# Autodesk Inventor assembly: mosaad pump
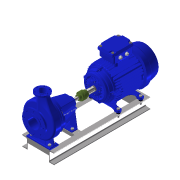
[picture p0: Inventor's stored thumbnail of the model, 180x180]
Saved by Autodesk Inventor 2016 (Build 200138000, 138)
## iProperties
Created: 2017-06-04
Part Number: mosaad pump
Document SubType Name: Assembly
Designer: Mohamed
Author: Mohamed
## Documents named in this file (12)
- C:\Users\Mohamed\Desktop\Mosaad pump\mosaad pump.iam
- C:\Users\Mohamed\Desktop\Mosaad pump\nnnnmmm.ipt
- C:\Users\Mohamed\Desktop\Mosaad pump\Assembly3.iam
- C:\Users\Mohamed\Desktop\Mosaad pump\DIN1026-1 - U 60 - 350.ipt
- C:\Users\Mohamed\Desktop\Mosaad pump\DIN1026-1 - U 80 - 350.ipt
- C:\Users\Mohamed\Desktop\Mosaad pump\rubber.ipt
- C:\Users\Mohamed\Documents\Inventor\Content Center Files\R2016\en-US\DIN 1026-1\DIN1026-1 - U 100 - 900.ipt
- C:\Users\Mohamed\Documents\Inventor\Content Center Files\R2016\en-US\DIN 933\DIN 933 - M14  x 65.ipt
- C:\Users\Mohamed\Documents\Inventor\Content Center Files\R2016\en-US\DIN 934\DIN 934 - M14 x 2.ipt
- C:\Users\Mohamed\Documents\Inventor\Content Center Files\R2016\en-US\DIN 1026-1\DIN1026-1 - U 100 - 200.ipt
- C:\Users\Mohamed\Desktop\Mosaad pump\coupling1.ipt
- C:\Users\Mohamed\Desktop\Mosaad pump\coupling2.ipt
## Components (27 placed, 11 different names)
1. nnnnmmm:1 — Mate:3, Angle:1, Mate:11, Mate:13, Mate:17, Mate:18, Mate:30, Mate:31, Mate:32, Mate:33, Mate:34, Mate:35, Mate:39, Mate:57, Mate:58
2. Assembly3:1 [sub-assembly] — Mate:3, Flush:6, Flush:8, Angle:1, Mate:24, Mate:25, Mate:41, Mate:42, Mate:43, Mate:44, Mate:45, Mate:46, Mate:47, Mate:48, Mate:49, Mate:50, Mate:51, Mate:52, Mate:59, Mate:60
3. DIN1026-1 - U 60 - 350:2 — Flush:7, Flush:8, Flush:12, Mate:27
4. DIN1026-1 - U 80 - 350:1 — Flush:6, Flush:7, Mate:22, Flush:13, Mate:24, Mate:26
5. rubber:1 — Mate:11, Mate:35
6. rubber:2 — Mate:17, Mate:33, Mate:54
7. rubber:3 — Mate:18, Mate:34, Mate:56
8. rubber:4 — Mate:13, Mate:32
9. DIN 1026-1 U 100 - 900:1 — Mate:26, Flush:14, Flush:15, Mate:40
10. DIN 1026-1 U 100 - 900:2 — Mate:22, Flush:12, Flush:13, Mate:23, Mate:25, Flush:14, Flush:15, Mate:27, Mate:36, Flush:18, Flush:19, Flush:24, Flush:25
11. DIN 933 - replaced by DIN EN 24017 M14  x 65:1 — Mate:30, Mate:31, Mate:37, Flush:16, Flush:20
12. DIN 934 - replaced by DIN EN 24032/28673/28674 M14:1 — Mate:36, Mate:37, Flush:17, Flush:21
13. DIN 933 - replaced by DIN EN 24017 M14  x 65:2 — Flush:16, Mate:39
14. DIN 934 - replaced by DIN EN 24032/28673/28674 M14:2 — Flush:17
15. DIN 1026-1 U 100 - 200:1 — Mate:40, Flush:18, Flush:19
16. DIN 933 - replaced by DIN EN 24017 M14  x 65:3 — Mate:41, Mate:42
17. DIN 933 - replaced by DIN EN 24017 M14  x 65:4 — Mate:43, Mate:44
18. DIN 933 - replaced by DIN EN 24017 M14  x 65:5 — Mate:45, Mate:46
19. DIN 933 - replaced by DIN EN 24017 M14  x 65:6 — Mate:47, Mate:48
20. DIN 933 - replaced by DIN EN 24017 M14  x 65:7 — Mate:49, Mate:50
21. DIN 933 - replaced by DIN EN 24017 M14  x 65:8 — Mate:51, Mate:52
22. DIN 933 - replaced by DIN EN 24017 M14  x 65:9 — Mate:54, Flush:20, Flush:23
23. DIN 934 - replaced by DIN EN 24032/28673/28674 M14:3 — Flush:21, Flush:22
24. DIN 933 - replaced by DIN EN 24017 M14  x 65:10 — Mate:56, Flush:23
25. DIN 934 - replaced by DIN EN 24032/28673/28674 M14:4 — Flush:22
26. coupling1:1 — Mate:57, Mate:58, Mate:61, Mate:62
27. coupling2:1 — Mate:59, Mate:60, Mate:61, Mate:62
## Relationships (62: Mate 44, Flush 17, Angle 1)
- Mate:3: nnnnmmm:1 ↔ Assembly3:1
- Flush:6: Assembly3:1 ↔ DIN1026-1 - U 80 - 350:1
- Flush:7: DIN1026-1 - U 60 - 350:2 ↔ DIN1026-1 - U 80 - 350:1
- Flush:8 (-3 mm): Assembly3:1 ↔ DIN1026-1 - U 60 - 350:2
- Angle:1 (0 deg): nnnnmmm:1 ↔ Assembly3:1
- Mate:11: nnnnmmm:1 ↔ rubber:1
- Mate:13: nnnnmmm:1 ↔ rubber:4
- Mate:17: nnnnmmm:1 ↔ rubber:2
- Mate:18: nnnnmmm:1 ↔ rubber:3
- Mate:22: DIN1026-1 - U 80 - 350:1 ↔ DIN 1026-1 U 100 - 900:2
- Flush:12: DIN1026-1 - U 60 - 350:2 ↔ DIN 1026-1 U 100 - 900:2
- Flush:13: DIN1026-1 - U 80 - 350:1 ↔ DIN 1026-1 U 100 - 900:2
- Mate:23: DIN 1026-1 U 100 - 900:2
- Mate:24: Assembly3:1 ↔ DIN1026-1 - U 80 - 350:1
- Mate:25 (-10 mm): Assembly3:1 ↔ DIN 1026-1 U 100 - 900:2
- Mate:26: DIN1026-1 - U 80 - 350:1 ↔ DIN 1026-1 U 100 - 900:1
- Flush:14: DIN 1026-1 U 100 - 900:1 ↔ DIN 1026-1 U 100 - 900:2
- Flush:15: DIN 1026-1 U 100 - 900:1 ↔ DIN 1026-1 U 100 - 900:2
- Mate:27: DIN1026-1 - U 60 - 350:2 ↔ DIN 1026-1 U 100 - 900:2
- Mate:30: nnnnmmm:1 ↔ DIN 933 - replaced by DIN EN 24017 M14  x 65:1
- Mate:31: nnnnmmm:1 ↔ DIN 933 - replaced by DIN EN 24017 M14  x 65:1
- Mate:32: nnnnmmm:1 ↔ rubber:4
- Mate:33: nnnnmmm:1 ↔ rubber:2
- Mate:34: nnnnmmm:1 ↔ rubber:3
- Mate:35: nnnnmmm:1 ↔ rubber:1
- Mate:36 (-20 mm): DIN 1026-1 U 100 - 900:2 ↔ DIN 934 - replaced by DIN EN 24032/28673/28674 M14:1
- Mate:37: DIN 933 - replaced by DIN EN 24017 M14  x 65:1 ↔ DIN 934 - replaced by DIN EN 24032/28673/28674 M14:1
- [Mate]: DIN 933 - replaced by DIN EN 24017 M14  x 65:2 ↔ DIN 934 - replaced by DIN EN 24032/28673/28674 M14:2
- Flush:16: DIN 933 - replaced by DIN EN 24017 M14  x 65:1 ↔ DIN 933 - replaced by DIN EN 24017 M14  x 65:2
- Mate:39: nnnnmmm:1 ↔ DIN 933 - replaced by DIN EN 24017 M14  x 65:2
- Flush:17: DIN 934 - replaced by DIN EN 24032/28673/28674 M14:1 ↔ DIN 934 - replaced by DIN EN 24032/28673/28674 M14:2
- Mate:40: DIN 1026-1 U 100 - 900:1 ↔ DIN 1026-1 U 100 - 200:1
- Flush:18: DIN 1026-1 U 100 - 900:2 ↔ DIN 1026-1 U 100 - 200:1
- Flush:19: DIN 1026-1 U 100 - 900:2 ↔ DIN 1026-1 U 100 - 200:1
- Mate:41: Assembly3:1 ↔ DIN 933 - replaced by DIN EN 24017 M14  x 65:3
- Mate:42: Assembly3:1 ↔ DIN 933 - replaced by DIN EN 24017 M14  x 65:3
- Mate:43: Assembly3:1 ↔ DIN 933 - replaced by DIN EN 24017 M14  x 65:4
- Mate:44: Assembly3:1 ↔ DIN 933 - replaced by DIN EN 24017 M14  x 65:4
- Mate:45: Assembly3:1 ↔ DIN 933 - replaced by DIN EN 24017 M14  x 65:5
- Mate:46: Assembly3:1 ↔ DIN 933 - replaced by DIN EN 24017 M14  x 65:5
- Mate:47: Assembly3:1 ↔ DIN 933 - replaced by DIN EN 24017 M14  x 65:6
- Mate:48: Assembly3:1 ↔ DIN 933 - replaced by DIN EN 24017 M14  x 65:6
- Mate:49: Assembly3:1 ↔ DIN 933 - replaced by DIN EN 24017 M14  x 65:7
- Mate:50: Assembly3:1 ↔ DIN 933 - replaced by DIN EN 24017 M14  x 65:7
- Mate:51: Assembly3:1 ↔ DIN 933 - replaced by DIN EN 24017 M14  x 65:8
- Mate:52: Assembly3:1 ↔ DIN 933 - replaced by DIN EN 24017 M14  x 65:8
- [Mate]: DIN 933 - replaced by DIN EN 24017 M14  x 65:9 ↔ DIN 934 - replaced by DIN EN 24032/28673/28674 M14:3
- Mate:54: rubber:2 ↔ DIN 933 - replaced by DIN EN 24017 M14  x 65:9
- Flush:20: DIN 933 - replaced by DIN EN 24017 M14  x 65:1 ↔ DIN 933 - replaced by DIN EN 24017 M14  x 65:9
- Flush:21: DIN 934 - replaced by DIN EN 24032/28673/28674 M14:1 ↔ DIN 934 - replaced by DIN EN 24032/28673/28674 M14:3
- [Mate]: DIN 933 - replaced by DIN EN 24017 M14  x 65:10 ↔ DIN 934 - replaced by DIN EN 24032/28673/28674 M14:4
- Mate:56: rubber:3 ↔ DIN 933 - replaced by DIN EN 24017 M14  x 65:10
- Flush:22: DIN 934 - replaced by DIN EN 24032/28673/28674 M14:3 ↔ DIN 934 - replaced by DIN EN 24032/28673/28674 M14:4
- Flush:23: DIN 933 - replaced by DIN EN 24017 M14  x 65:9 ↔ DIN 933 - replaced by DIN EN 24017 M14  x 65:10
- Mate:57: nnnnmmm:1 ↔ coupling1:1
- Mate:58 (-15 mm): nnnnmmm:1 ↔ coupling1:1
- Mate:59: Assembly3:1 ↔ coupling2:1
- Mate:60 (-15 mm): Assembly3:1 ↔ coupling2:1
- Mate:61: coupling1:1 ↔ coupling2:1
- Mate:62: coupling1:1 ↔ coupling2:1
- Flush:24 (-450 mm): DIN 1026-1 U 100 - 900:2
- Flush:25 (-150 mm): DIN 1026-1 U 100 - 900:2
## Named parameters: d64_d63 = 0 mm, d83_d63 = 0 mm, d87_d83_d63 = 0 mm
